# Autodesk Inventor assembly: phalanx_plate
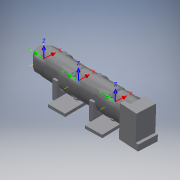
[picture p0: Inventor's stored thumbnail of the model, 180x180]
Saved by Autodesk Inventor 2019 (Build 230136000, 136)
## iProperties
Created: 2024-08-23
Part Number: phalanx_plate
Material: Generisch
Document SubType Name: Assembly
Designer: nic
Author: nic
## Documents named in this file (5)
- C:\Users\Nicolas Frick\Sync\OneDrive\wtm\nicol_rh8d\inventor\phalanx_plate.iam
- C:\Users\Nicolas Frick\Sync\OneDrive\wtm\nias\nias_description\inventor_files\hand\r_rh8d_refac\phalanx_refac.ipt
- C:\Users\Nicolas Frick\Sync\OneDrive\wtm\nicol_rh8d\inventor\phalanx_plate.ipt
- C:\Users\Nicolas Frick\Sync\OneDrive\wtm\nias\nias_description\inventor_files\hand\r_rh8d_refac\tip_refac.ipt
- C:\Users\Nicolas Frick\Sync\OneDrive\wtm\nicol_rh8d\inventor\tip_plate.ipt
## Components (6 placed, 4 different names)
1. phalanx_refac:1 — Fluchtend:2, Fluchtend:4, Passend:3, Passend:4, Passend:5, Passend:7, Fluchtend:5, Passend:8, Passend:9
2. phalanx_plate:1 — Fluchtend:2, Fluchtend:4, Passend:7, Fluchtend:5
3. phalanx_refac:2 — Passend:3, Passend:4, Passend:6
4. tip_refac:1 — Passend:8, Passend:9, Fluchtend:6, Fluchtend:7, Fluchtend:8
5. phalanx_plate:2 — Passend:5, Passend:6
6. tip_plate:1 — Fluchtend:6, Fluchtend:7, Fluchtend:8
## Relationships (13: Mate 7, Flush 6)
- Fluchtend:2 [Flush]: phalanx_refac:1 ↔ phalanx_plate:1
- Fluchtend:4 [Flush] (-3.5 mm): phalanx_refac:1 ↔ phalanx_plate:1
- Passend:3 [Mate]: phalanx_refac:1 ↔ phalanx_refac:2
- Passend:4 [Mate] (0.8 mm): phalanx_refac:1 ↔ phalanx_refac:2
- Passend:5 [Mate]: phalanx_refac:1 ↔ phalanx_plate:2
- Passend:6 [Mate] (0.2 mm): phalanx_refac:2 ↔ phalanx_plate:2
- Passend:7 [Mate]: phalanx_refac:1 ↔ phalanx_plate:1
- Fluchtend:5 [Flush] (3.5 mm): phalanx_refac:1 ↔ phalanx_plate:1
- Passend:8 [Mate]: phalanx_refac:1 ↔ tip_refac:1
- Passend:9 [Mate] (0.8 mm): phalanx_refac:1 ↔ tip_refac:1
- Fluchtend:6 [Flush]: tip_refac:1 ↔ tip_plate:1
- Fluchtend:7 [Flush]: tip_refac:1 ↔ tip_plate:1
- Fluchtend:8 [Flush]: tip_refac:1 ↔ tip_plate:1
